# Autodesk Inventor assembly: BaseSuperior
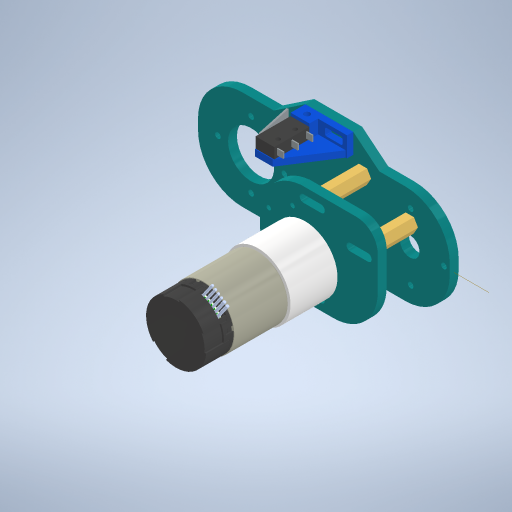
[picture p0: Inventor's stored thumbnail of the model, 512x512]
Saved by Autodesk Inventor 2024.3 (Build 283343000, 343)
## iProperties
Created: 2024-09-30
Part Number: BaseSuperior
Document SubType Name: Assembly
Designer: User
Author: User
## Documents named in this file (6)
- C:\Users\User\Documents\Universidad Octavo Semestre\Robotica Industrial\matlab\SCARA\mariana_scara_final\mariana_scara_final\BaseSuperior.iam
- C:\Users\User\Documents\Universidad Octavo Semestre\Robotica Industrial\matlab\SCARA\mariana_scara_final\mariana_scara_final\lamina_superior.ipt
- C:\Users\User\Documents\Universidad Octavo Semestre\Robotica Industrial\matlab\SCARA\mariana_scara_final\mariana_scara_final\separador.ipt
- C:\Users\User\Documents\Universidad Octavo Semestre\Robotica Industrial\matlab\SCARA\mariana_scara_final\mariana_scara_final\final_carrera.iam
- C:\Users\User\Documents\Universidad Octavo Semestre\Robotica Industrial\matlab\SCARA\mariana_scara_final\mariana_scara_final\lamina_motor_superior.ipt
- C:\Users\User\Documents\Universidad Octavo Semestre\Robotica Industrial\matlab\SCARA\mariana_scara_final\mariana_scara_final\motor_1.ipt
## Components (8 placed, 5 different names)
1. lamina_superior:1 — Mate:1, Mate:2, Mate:3, Mate:4, Mate:5, Mate:6, Flush:1, Mate:7, Mate:8, Flush:2, Mate:9, Mate:10, Flush:3, Flush:4
2. separador:1 — Mate:1, Mate:2, Angle:1, Angle:2
3. separador:2 — Mate:3, Mate:4, Angle:2, Angle:3
4. separador:3 — Mate:5, Mate:6, Angle:3, Mate:11
5. final_carrera:1 [sub-assembly] — Flush:1, Mate:7, Mate:8
6. final_carrera:2 [sub-assembly] — Flush:2, Mate:9, Mate:10
7. lamina_motor_superior:1 — Mate:11, Flush:3, Flush:4, Insert:1
8. motor_1:1 — Insert:1
## Relationships (19: Mate 11, Flush 4, Angle 3, Insert 1)
- Mate:1: lamina_superior:1 ↔ separador:1
- Mate:2: lamina_superior:1 ↔ separador:1
- Angle:1 (90 deg): separador:1
- Mate:3: lamina_superior:1 ↔ separador:2
- Mate:4: lamina_superior:1 ↔ separador:2
- Angle:2 (0 deg): separador:1 ↔ separador:2
- Mate:5: lamina_superior:1 ↔ separador:3
- Mate:6: lamina_superior:1 ↔ separador:3
- Angle:3 (0 deg): separador:2 ↔ separador:3
- Flush:1: lamina_superior:1 ↔ final_carrera:1
- Mate:7: lamina_superior:1 ↔ final_carrera:1
- Mate:8: lamina_superior:1 ↔ final_carrera:1
- Flush:2: lamina_superior:1 ↔ final_carrera:2
- Mate:9: lamina_superior:1 ↔ final_carrera:2
- Mate:10: lamina_superior:1 ↔ final_carrera:2
- Mate:11: separador:3 ↔ lamina_motor_superior:1
- Flush:3 (12 mm): lamina_superior:1 ↔ lamina_motor_superior:1
- Flush:4 (12 mm): lamina_superior:1 ↔ lamina_motor_superior:1
- Insert:1: lamina_motor_superior:1 ↔ motor_1:1
